# Autodesk Inventor assembly: sod_ii_complete
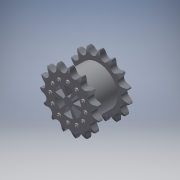
[picture p0: Inventor's stored thumbnail of the model, 180x180]
Saved by Autodesk Inventor 2016 (Build 200138000, 138)
## iProperties
Created: 2016-11-20
Part Number: sod_ii_complete
Document SubType Name: Assembly
Designer: hesaon
Author: hesaon
## Documents named in this file (6)
- D:\documents\SOD-II\cad\sod_ii_complete.iam
- D:\documents\SOD-II\cad\drive_sprocket_middle.ipt
- D:\documents\SOD-II\cad\outer_drive_sprocket.ipt
- D:\documents\SOD-II\cad\screw_Ka22x16.ipt
- D:\documents\SOD-II\cad\motor_axle_mounting_hub_6_mm.ipt
- D:\documents\SOD-II\cad\drive_sprocket_inner.ipt
## Components (16 placed, 5 different names)
1. drive_sprocket_middle:1 — Insert:1, Insert:2, Insert:16, Insert:17
2. outer_drive_sprocket:1 — Insert:1, Insert:2, Insert:3, Insert:4, Insert:5, Insert:6, Insert:7, Insert:8, Insert:9, Insert:10, Insert:11, Insert:12, Insert:13, Insert:14
3. screw_Ka22x16:1 — Insert:6
4. screw_Ka22x16:2 — Insert:4
5. screw_Ka22x16:3 — Insert:3
6. screw_Ka22x16:4 — Insert:7
7. screw_Ka22x16:5 — Insert:10
8. screw_Ka22x16:6 — Insert:9
9. screw_Ka22x16:7 — Insert:8
10. screw_Ka22x16:8 — Insert:5
11. screw_Ka22x16:9 — Insert:14
12. screw_Ka22x16:10 — Insert:11
13. screw_Ka22x16:11 — Insert:12
14. screw_Ka22x16:12 — Insert:13
15. motor_axle_mounting_hub_6_mm:1 — Insert:15, Mate:1
16. drive_sprocket_inner:1 — Insert:15, Mate:1, Insert:16, Insert:17
## Relationships (18: Insert 17, Mate 1)
- Insert:1: drive_sprocket_middle:1 ↔ outer_drive_sprocket:1
- Insert:2: drive_sprocket_middle:1 ↔ outer_drive_sprocket:1
- Insert:3: outer_drive_sprocket:1 ↔ screw_Ka22x16:3
- Insert:4: outer_drive_sprocket:1 ↔ screw_Ka22x16:2
- Insert:5: outer_drive_sprocket:1 ↔ screw_Ka22x16:8
- Insert:6: outer_drive_sprocket:1 ↔ screw_Ka22x16:1
- Insert:7: outer_drive_sprocket:1 ↔ screw_Ka22x16:4
- Insert:8: outer_drive_sprocket:1 ↔ screw_Ka22x16:7
- Insert:9: outer_drive_sprocket:1 ↔ screw_Ka22x16:6
- Insert:10: outer_drive_sprocket:1 ↔ screw_Ka22x16:5
- Insert:11: outer_drive_sprocket:1 ↔ screw_Ka22x16:10
- Insert:12: outer_drive_sprocket:1 ↔ screw_Ka22x16:11
- Insert:13: outer_drive_sprocket:1 ↔ screw_Ka22x16:12
- Insert:14: outer_drive_sprocket:1 ↔ screw_Ka22x16:9
- Insert:15: motor_axle_mounting_hub_6_mm:1 ↔ drive_sprocket_inner:1
- Mate:1: motor_axle_mounting_hub_6_mm:1 ↔ drive_sprocket_inner:1
- Insert:16: drive_sprocket_middle:1 ↔ drive_sprocket_inner:1
- Insert:17: drive_sprocket_middle:1 ↔ drive_sprocket_inner:1
